# Autodesk Inventor assembly: Ball_05mm Blue
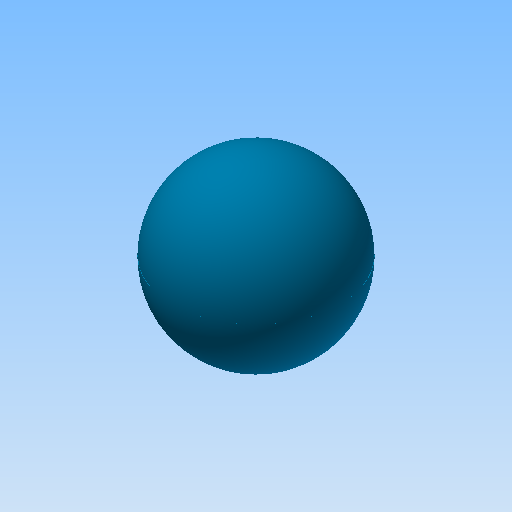
[picture p0: Inventor's stored thumbnail of the model, 512x512]
Saved by Autodesk Inventor 2018.1 (Build 221171000, 171)
## iProperties
Created: 2019-03-22
Part Number: Ball_05mm Blue
Document SubType Name: Assembly
Designer: James
Author: James
## Documents named in this file (3)
- C:\Users\admin\Desktop\Ball-Machine\Balls\Ball_05mm Blue.iam
- C:\Users\admin\Desktop\Ball-Machine\Balls\Ball_Half Sphere 5.ipt
- C:\Users\admin\Desktop\Ball-Machine\Balls\Steel Ball 05mm.ipt
## Components (3 placed, 2 different names)
1. Ball_Half Sphere 5:1 — Flush:1, Flush:2, Flush:3, Tangent:1, Mate:1, Mate:2
2. Steel Ball 05mm:1 — Tangent:1
3. Ball_Half Sphere 5:2 — Mate:1, Mate:2
## Relationships (6: Flush 3, Mate 2, Tangent 1)
- Flush:1: Ball_Half Sphere 5:1
- Flush:2: Ball_Half Sphere 5:1
- Flush:3: Ball_Half Sphere 5:1
- Tangent:1 (-0.5 mm): Ball_Half Sphere 5:1 ↔ Steel Ball 05mm:1
- Mate:1: Ball_Half Sphere 5:1 ↔ Ball_Half Sphere 5:2
- Mate:2: Ball_Half Sphere 5:1 ↔ Ball_Half Sphere 5:2
